# Autodesk Inventor assembly: nasel_poalset2
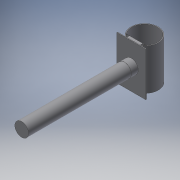
[picture p0: Inventor's stored thumbnail of the model, 180x180]
Saved by Autodesk Inventor 2016 SP1 (Build 200210100, 210)
## iProperties
Created: 2017-01-27
Part Number: nasel_poalset2
Material: 一般
Document SubType Name: Assembly
Designer: p_admin
Author: p_admin
## Documents named in this file (4)
- Z:\風力発電機\nasel_poalset2.iam
- Z:\風力発電機\poal1.ipt
- Z:\風力発電機\nasel_stand.ipt
- Z:\風力発電機\nasel2.ipt
## Components (3 placed, 3 different names)
1. poal1:1 — リジッド:1
2. nasel_stand:1 — フラッシュ:1, スライダ:1, リジッド:1
3. nasel2:1 — フラッシュ:1, スライダ:1
## Relationships (3: Flush 1, TranslationJoint 1, WeldJoint 1)
- フラッシュ:1 [Flush]: nasel_stand:1 ↔ nasel2:1
- スライダ:1 [TranslationJoint]: nasel_stand:1 ↔ nasel2:1
- リジッド:1 [WeldJoint]: poal1:1 ↔ nasel_stand:1
